# Autodesk Inventor assembly: сборка полностью свободной шестерни
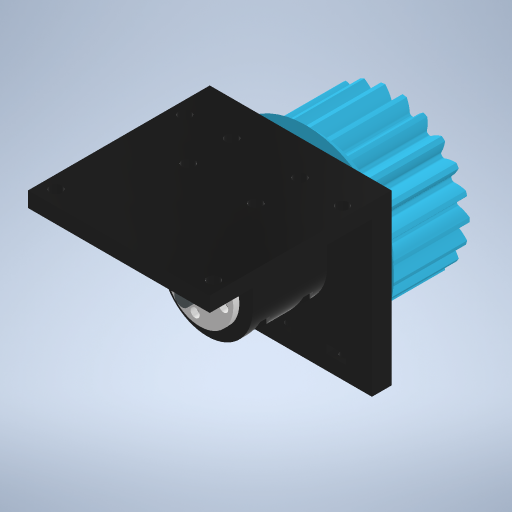
[picture p0: Inventor's stored thumbnail of the model, 512x512]
Saved by Autodesk Inventor 2024.2 (Build 282272000, 272)
## iProperties
Created: 2026-01-30
Part Number: сборка полностью свободной шестерни
Document SubType Name: Assembly
Designer: katya_notebook
Author: katya_notebook
## Documents named in this file (7)
- D:\alletz\construction\сборка полностью свободной шестерни.iam
- D:\alletz\construction\крепление свободной шестерни.ipt
- D:\alletz\construction\верх штуки для подшипников.ipt
- D:\alletz\construction\подшипник.ipt
- D:\alletz\construction\муфта.ipt
- D:\alletz\construction\вал.ipt
- D:\alletz\construction\шестерня версия 3.ipt
## Components (9 placed, 6 different names)
1. крепление свободной шестерни:1 — Цилиндрический:1, Совмещение:2, Совмещение:3, Совмещение:4
2. верх штуки для подшипников:1 — Совмещение:3, Совмещение:4
3. подшипник:1 — Цилиндрический:1, Совмещение:2, С поворотом:1, С поворотом:6
4. подшипник:2 — С поворотом:1, С поворотом:2
5. подшипник:3 — С поворотом:2, С поворотом:4
6. муфта:1 — С поворотом:4
7. вал:1 — С поворотом:7
8. шестерня версия 3:1 — С поворотом:5, Совмещение:5, С поворотом:7
9. муфта:2 — С поворотом:5, Совмещение:5, С поворотом:6
## Relationships (11: RevoluteJoint 6, Mate 4, CylindricalJoint 1)
- Цилиндрический:1 [CylindricalJoint]: крепление свободной шестерни:1 ↔ подшипник:1
- Совмещение:2 [Mate]: крепление свободной шестерни:1 ↔ подшипник:1
- С поворотом:1 [RevoluteJoint]: подшипник:1 ↔ подшипник:2
- С поворотом:2 [RevoluteJoint]: подшипник:2 ↔ подшипник:3
- С поворотом:4 [RevoluteJoint]: подшипник:3 ↔ муфта:1
- Совмещение:3 [Mate]: крепление свободной шестерни:1 ↔ верх штуки для подшипников:1
- Совмещение:4 [Mate]: крепление свободной шестерни:1 ↔ верх штуки для подшипников:1
- С поворотом:5 [RevoluteJoint]: шестерня версия 3:1 ↔ муфта:2
- Совмещение:5 [Mate]: шестерня версия 3:1 ↔ муфта:2
- С поворотом:6 [RevoluteJoint]: подшипник:1 ↔ муфта:2
- С поворотом:7 [RevoluteJoint]: вал:1 ↔ шестерня версия 3:1
